# Autodesk Inventor assembly: Trash_Storage_Unit
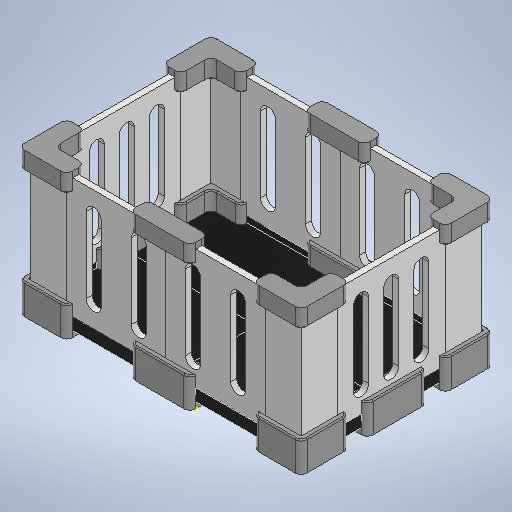
[picture p0: Inventor's stored thumbnail of the model, 512x512]
Saved by Autodesk Inventor 2025.2 (Build 292293000, 293)
## iProperties
Created: 2025-01-07
Part Number: Trash_Storage_Unit
Document SubType Name: Assembly
Designer: Matt Tidd
Author: Matt Tidd
## Documents named in this file (11)
- C:\Users\mtidd2\Desktop\H2A\CAD\TrashStorageUnit\Trash_Storage_Unit.iam
- C:\Users\mtidd2\Desktop\H2A\CAD\TrashStorageUnit\TSU_FM_Floor.ipt
- C:\Users\mtidd2\Desktop\H2A\CAD\TrashStorageUnit\TSU_MF_Floor.ipt
- C:\Users\mtidd2\Desktop\H2A\CAD\TrashStorageUnit\TSU_Y_Clamp.ipt
- C:\Users\mtidd2\Desktop\H2A\CAD\TrashStorageUnit\TSU_FF_Corner_Wall.ipt
- C:\Users\mtidd2\Desktop\H2A\CAD\TrashStorageUnit\TSU_MM_Wall.ipt
- C:\Users\mtidd2\Desktop\H2A\CAD\TrashStorageUnit\TSU_FM_Side_Wall.ipt
- C:\Users\mtidd2\Desktop\H2A\CAD\TrashStorageUnit\TSU_MM_Side_Wall.ipt
- C:\Users\mtidd2\Desktop\H2A\CAD\TrashStorageUnit\TSU_Corner_Clamp.ipt
- C:\Users\mtidd2\Desktop\H2A\CAD\TrashStorageUnit\TSU_Corner_Top_Clamp.ipt
- C:\Users\mtidd2\Desktop\H2A\CAD\TrashStorageUnit\TSU_Middle_Top_Clamp.ipt
## Components (28 placed, 10 different names)
1. TSU_FM_Floor:1 — Mate:5, Mate:6, Mate:7, Mate:8, Mate:21, Mate:22
2. TSU_MF_Floor:1 — Mate:3, Mate:4, Mate:9, Mate:10, Mate:16
3. TSU_FM_Floor:2 — Mate:1, Mate:2, Mate:3, Mate:4, Mate:13, Mate:14, Mate:15, Mate:17, Mate:18
4. TSU_MF_Floor:2 — Mate:1, Mate:2, Mate:5, Mate:6, Mate:11, Mate:12, Mate:19, Mate:20
5. TSU_Corner_Clamp:1 — Mate:9, Mate:10, Mate:25, Mate:26
6. TSU_Corner_Clamp:2 — Mate:13, Mate:14
7. TSU_Corner_Clamp:3 — Mate:11, Mate:12, Mate:27, Mate:28
8. TSU_Corner_Clamp:4 — Mate:7, Mate:8, Mate:23, Mate:24
9. TSU_Y_Clamp:1 — Mate:19, Mate:20
10. TSU_Y_Clamp:2 — Mate:17, Mate:18
11. TSU_Y_Clamp:3 — Mate:15, Mate:16
12. TSU_Y_Clamp:4 — Mate:21, Mate:22
13. TSU_FF_Corner_Wall:1 — Mate:23, Mate:24, Mate:31, Mate:32, Mate:45
14. TSU_FF_Corner_Wall:2 — Mate:25, Mate:26, Mate:33, Mate:34, Mate:41, Mate:42, Mate:43
15. TSU_FF_Corner_Wall:3 — Mate:47
16. TSU_FF_Corner_Wall:4 — Mate:27, Mate:28, Mate:39, Mate:40, Mate:49, Mate:50
17. TSU_FM_Side_Wall:1 — Mate:31, Mate:32, Mate:35, Mate:36, Mate:46
18. TSU_FM_Side_Wall:2 — Mate:33, Mate:34, Mate:37, Mate:44, Mate:54
19. TSU_MM_Side_Wall:1 — Mate:35, Mate:36, Mate:51, Mate:52
20. TSU_MM_Side_Wall:2 — Mate:37, Mate:53
21. TSU_MM_Wall:1 — Mate:41, Mate:42
22. TSU_MM_Wall:2 — Mate:39, Mate:40, Mate:48
23. TSU_Corner_Top_Clamp:1 — Mate:45, Mate:46
24. TSU_Corner_Top_Clamp:2 — Mate:49, Mate:50
25. TSU_Corner_Top_Clamp:3 — Mate:47, Mate:48
26. TSU_Corner_Top_Clamp:4 — Mate:43, Mate:44
27. TSU_Middle_Top_Clamp:1 — Mate:51, Mate:52
28. TSU_Middle_Top_Clamp:2 — Mate:53, Mate:54
## Relationships (51: Mate 51)
- Mate:1: TSU_FM_Floor:2 ↔ TSU_MF_Floor:2
- Mate:2: TSU_FM_Floor:2 ↔ TSU_MF_Floor:2
- Mate:3: TSU_MF_Floor:1 ↔ TSU_FM_Floor:2
- Mate:4: TSU_MF_Floor:1 ↔ TSU_FM_Floor:2
- Mate:5: TSU_FM_Floor:1 ↔ TSU_MF_Floor:2
- Mate:6: TSU_FM_Floor:1 ↔ TSU_MF_Floor:2
- Mate:7: TSU_FM_Floor:1 ↔ TSU_Corner_Clamp:4
- Mate:8: TSU_FM_Floor:1 ↔ TSU_Corner_Clamp:4
- Mate:9: TSU_MF_Floor:1 ↔ TSU_Corner_Clamp:1
- Mate:10: TSU_MF_Floor:1 ↔ TSU_Corner_Clamp:1
- Mate:11: TSU_MF_Floor:2 ↔ TSU_Corner_Clamp:3
- Mate:12: TSU_MF_Floor:2 ↔ TSU_Corner_Clamp:3
- Mate:13: TSU_FM_Floor:2 ↔ TSU_Corner_Clamp:2
- Mate:14: TSU_FM_Floor:2 ↔ TSU_Corner_Clamp:2
- Mate:15: TSU_FM_Floor:2 ↔ TSU_Y_Clamp:3
- Mate:16: TSU_MF_Floor:1 ↔ TSU_Y_Clamp:3
- Mate:17: TSU_FM_Floor:2 ↔ TSU_Y_Clamp:2
- Mate:18: TSU_FM_Floor:2 ↔ TSU_Y_Clamp:2
- Mate:19: TSU_MF_Floor:2 ↔ TSU_Y_Clamp:1
- Mate:20: TSU_MF_Floor:2 ↔ TSU_Y_Clamp:1
- Mate:21: TSU_FM_Floor:1 ↔ TSU_Y_Clamp:4
- Mate:22: TSU_FM_Floor:1 ↔ TSU_Y_Clamp:4
- Mate:23: TSU_Corner_Clamp:4 ↔ TSU_FF_Corner_Wall:1
- Mate:24: TSU_Corner_Clamp:4 ↔ TSU_FF_Corner_Wall:1
- Mate:25: TSU_Corner_Clamp:1 ↔ TSU_FF_Corner_Wall:2
- Mate:26: TSU_Corner_Clamp:1 ↔ TSU_FF_Corner_Wall:2
- Mate:27: TSU_Corner_Clamp:3 ↔ TSU_FF_Corner_Wall:4
- Mate:28: TSU_Corner_Clamp:3 ↔ TSU_FF_Corner_Wall:4
- Mate:31: TSU_FF_Corner_Wall:1 ↔ TSU_FM_Side_Wall:1
- Mate:32: TSU_FF_Corner_Wall:1 ↔ TSU_FM_Side_Wall:1
- Mate:33: TSU_FF_Corner_Wall:2 ↔ TSU_FM_Side_Wall:2
- Mate:34: TSU_FF_Corner_Wall:2 ↔ TSU_FM_Side_Wall:2
- Mate:35: TSU_FM_Side_Wall:1 ↔ TSU_MM_Side_Wall:1
- Mate:36: TSU_FM_Side_Wall:1 ↔ TSU_MM_Side_Wall:1
- Mate:37: TSU_FM_Side_Wall:2 ↔ TSU_MM_Side_Wall:2
- Mate:39: TSU_FF_Corner_Wall:4 ↔ TSU_MM_Wall:2
- Mate:40: TSU_FF_Corner_Wall:4 ↔ TSU_MM_Wall:2
- Mate:41: TSU_FF_Corner_Wall:2 ↔ TSU_MM_Wall:1
- Mate:42: TSU_FF_Corner_Wall:2 ↔ TSU_MM_Wall:1
- Mate:43: TSU_FF_Corner_Wall:2 ↔ TSU_Corner_Top_Clamp:4
- Mate:44: TSU_FM_Side_Wall:2 ↔ TSU_Corner_Top_Clamp:4
- Mate:45: TSU_FF_Corner_Wall:1 ↔ TSU_Corner_Top_Clamp:1
- Mate:46: TSU_FM_Side_Wall:1 ↔ TSU_Corner_Top_Clamp:1
- Mate:47: TSU_FF_Corner_Wall:3 ↔ TSU_Corner_Top_Clamp:3
- Mate:48: TSU_MM_Wall:2 ↔ TSU_Corner_Top_Clamp:3
- Mate:49: TSU_FF_Corner_Wall:4 ↔ TSU_Corner_Top_Clamp:2
- Mate:50: TSU_FF_Corner_Wall:4 ↔ TSU_Corner_Top_Clamp:2
- Mate:51: TSU_MM_Side_Wall:1 ↔ TSU_Middle_Top_Clamp:1
- Mate:52: TSU_MM_Side_Wall:1 ↔ TSU_Middle_Top_Clamp:1
- Mate:53: TSU_MM_Side_Wall:2 ↔ TSU_Middle_Top_Clamp:2
- Mate:54: TSU_FM_Side_Wall:2 ↔ TSU_Middle_Top_Clamp:2
